# Autodesk Inventor assembly: structure_channel_mirrored
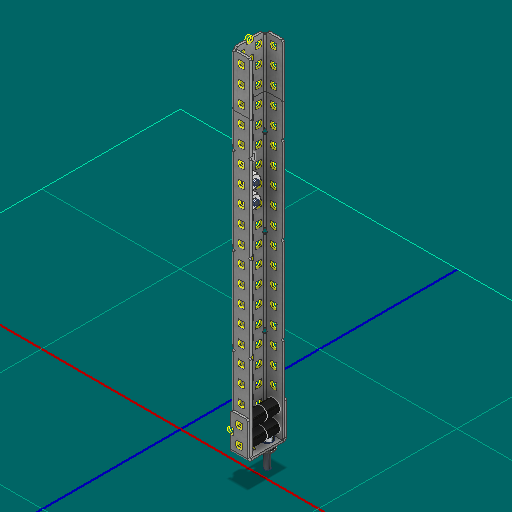
[picture p0: Inventor's stored thumbnail of the model, 512x512]
Saved by Autodesk Inventor 2025 (Build 290162000, 162)
## iProperties
Created: 2024-08-18
Part Number: structure_channel_mirrored
Document SubType Name: Assembly
Designer: averey
Author: averey
## Documents named in this file (14)
- C:\Users\avere\vex_robotics_high_stakes\hardware\cad\ATLAS\tower\structure\structure_channel_mirrored\structure_channel_mirrored.iam
- C:\Users\avere\vex_robotics_high_stakes\hardware\cad\ATLAS\tower\structure\structure_channel_mirrored\Alu C 1x2x1x20_mirrored.ipt
- C:\Users\avere\vex_robotics_high_stakes\hardware\cad\ATLAS\tower\structure\structure_channel_mirrored\Alu C 2x2x2x1_mirrored.ipt
- C:\Users\avere\vex_robotics_high_stakes\hardware\cad\VEX-CAD-Inventor\Motion\Spacers\Spacer Nylon .375 OD\NSpacer .375 OD x .375.ipt
- C:\Users\avere\vex_robotics_high_stakes\hardware\cad\VEX-CAD-Inventor\Motion\Spacers\Spacer Nylon .375 OD.ipt
- C:\Users\avere\vex_robotics_high_stakes\hardware\cad\VEX-CAD-Inventor\Motion\Spacers\Spacer Nylon .375 OD\NSpacer .375 OD x .500.ipt
- C:\Users\avere\vex_robotics_high_stakes\hardware\cad\VEX-CAD-Inventor\Structure\C Channel\Aluminum 1x2x1\Alu C 1x2x1x17.ipt
- C:\Users\avere\vex_robotics_high_stakes\hardware\cad\VEX-CAD-Inventor\Structure\Hardware\Screw Steel - Star\SScrew Star Smooth .750.ipt
- C:\Users\avere\vex_robotics_high_stakes\hardware\cad\VEX-CAD-Inventor\Structure\Hardware\Screw Steel - Star.ipt
- C:\Users\avere\vex_robotics_high_stakes\hardware\cad\VEX-CAD-Inventor\Motion\Spacers\Spacer Nylon .375 OD\NSpacer .375 OD x .125.ipt
- C:\Users\avere\vex_robotics_high_stakes\hardware\cad\VEX-CAD-Inventor\Motion\Spacers\Washer Steel\SWasher .375 OD x .015625.ipt
- C:\Users\avere\vex_robotics_high_stakes\hardware\cad\VEX-CAD-Inventor\Motion\Spacers\Washer Steel.ipt
- C:\Users\avere\vex_robotics_high_stakes\hardware\cad\VEX-CAD-Inventor\Motion\Spacers\Washer Steel\SWasher .375 OD x .031250.ipt
- C:\Users\avere\vex_robotics_high_stakes\hardware\cad\_quick_assemblies\bearing_flat_w_hardware_offset.iam
## Components (12 placed, 10 different names)
1. Alu C 1x2x1x20_mirrored:1 — Mate:5, Angle:2, Angle:1, Mate:6, Insert:1, Insert:3, Insert:5
2. Alu C 2x2x2x1_mirrored:1 — Mate:6, Insert:1, Insert:6, Mate:3, Insert:7, Insert:8
3. NSpacer .375 OD x .375:1 — Insert:2
4. NSpacer .375 OD x .500:2 — Insert:3, Insert:2
5. NSpacer .375 OD x .375:3 — Insert:4
6. NSpacer .375 OD x .500:4 — Insert:5, Insert:4
7. Alu C 1x2x1x17:1 — Insert:6, Mate:3, Insert:11, Mate:4
8. SScrew Star Smooth .750:1 — Insert:7
9. NSpacer .375 OD x .125:5 — Insert:8, Insert:10
10. SWasher .375 OD x .015625:1 — Insert:9
11. SWasher .375 OD x .031250:2 — Insert:9, Insert:10
12. bearing_flat_w_hardware_offset:1 [sub-assembly] — Insert:11, Mate:4
## Relationships (17: Insert 11, Mate 4, Angle 2)
- Mate:5 (49.6316 mm): Alu C 1x2x1x20_mirrored:1
- Angle:2 (0 deg): Alu C 1x2x1x20_mirrored:1
- Angle:1 (0 deg): Alu C 1x2x1x20_mirrored:1
- Mate:6: Alu C 1x2x1x20_mirrored:1 ↔ Alu C 2x2x2x1_mirrored:1
- Insert:1: Alu C 1x2x1x20_mirrored:1 ↔ Alu C 2x2x2x1_mirrored:1
- Insert:3: Alu C 1x2x1x20_mirrored:1 ↔ NSpacer .375 OD x .500:2
- Insert:2: NSpacer .375 OD x .375:1 ↔ NSpacer .375 OD x .500:2
- Insert:5: Alu C 1x2x1x20_mirrored:1 ↔ NSpacer .375 OD x .500:4
- Insert:4: NSpacer .375 OD x .375:3 ↔ NSpacer .375 OD x .500:4
- Insert:6: Alu C 2x2x2x1_mirrored:1 ↔ Alu C 1x2x1x17:1
- Mate:3: Alu C 2x2x2x1_mirrored:1 ↔ Alu C 1x2x1x17:1
- Insert:7: Alu C 2x2x2x1_mirrored:1 ↔ SScrew Star Smooth .750:1
- Insert:8: Alu C 2x2x2x1_mirrored:1 ↔ NSpacer .375 OD x .125:5
- Insert:9: SWasher .375 OD x .015625:1 ↔ SWasher .375 OD x .031250:2
- Insert:10: NSpacer .375 OD x .125:5 ↔ SWasher .375 OD x .031250:2
- Insert:11: Alu C 1x2x1x17:1 ↔ bearing_flat_w_hardware_offset:1
- Mate:4: Alu C 1x2x1x17:1 ↔ bearing_flat_w_hardware_offset:1
